# Autodesk Inventor assembly: FullFrontFrame
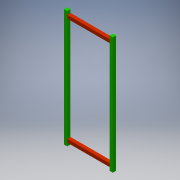
[picture p0: Inventor's stored thumbnail of the model, 180x180]
Saved by Autodesk Inventor 2019 (Build 230136000, 136)
## iProperties
Created: 2019-01-09
Part Number: FullFrontFrame
Document SubType Name: Assembly
Designer: james
Author: james
## Documents named in this file (3)
- F:\JimsDesign\2019CHS4089\FullFrontFrame.iam
- F:\JimsDesign\2019CHS4089\FrontBeam.ipt
- F:\JimsDesign\2019CHS4089\CrossBeam.ipt
## Components (4 placed, 2 different names)
1. FrontBeam:1 — Mate:1, Flush:1, Flush:2, Mate:3, Flush:5, Flush:6
2. FrontBeam:2 — Mate:2, Flush:3, Flush:4
3. CrossBeam:1 — Mate:1, Flush:1, Flush:2, Mate:2, Flush:3, Flush:4
4. CrossBeam:2 — Mate:3, Flush:5, Flush:6
## Relationships (9: Flush 6, Mate 3)
- Mate:1: FrontBeam:1 ↔ CrossBeam:1
- Flush:1: FrontBeam:1 ↔ CrossBeam:1
- Flush:2 (-25.4 mm): FrontBeam:1 ↔ CrossBeam:1
- Mate:2: FrontBeam:2 ↔ CrossBeam:1
- Flush:3: FrontBeam:2 ↔ CrossBeam:1
- Flush:4 (25.4 mm): FrontBeam:2 ↔ CrossBeam:1
- Mate:3: FrontBeam:1 ↔ CrossBeam:2
- Flush:5: FrontBeam:1 ↔ CrossBeam:2
- Flush:6 (-25.4 mm): FrontBeam:1 ↔ CrossBeam:2
